# Autodesk Inventor assembly: 04-3
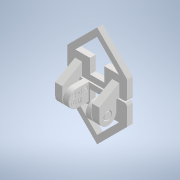
[picture p0: Inventor's stored thumbnail of the model, 180x180]
Saved by Autodesk Inventor 2022 (Build 260153000, 153)
## iProperties
Created: 2021-09-12
Part Number: 04-3
Document SubType Name: Assembly
Designer: 서울공업고등학교
Author: 서울공업고등학교
## Documents named in this file (3)
- C:\Users\서울공업고등학교\Documents\_9_12\모의고사9\04-3.iam
- C:\Users\서울공업고등학교\Documents\_9_12\모의고사9\01-1.ipt
- C:\Users\서울공업고등학교\Documents\_9_12\모의고사9\02-2.ipt
## Components (2 placed, 2 different names)
1. 01-1:1 — 메이트:1, 메이트:2, 각도:1
2. 02-2:1 — 메이트:1, 메이트:2, 각도:1
## Relationships (3: Mate 2, Angle 1)
- 메이트:1 [Mate]: 01-1:1 ↔ 02-2:1
- 메이트:2 [Mate] (0.5 mm): 01-1:1 ↔ 02-2:1
- 각도:1 [Angle] (180 deg): 01-1:1 ↔ 02-2:1
